# Autodesk Inventor assembly: for_bool
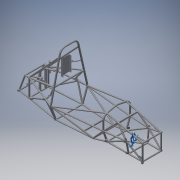
[picture p0: Inventor's stored thumbnail of the model, 180x180]
Saved by Autodesk Inventor 2018 (Build 220112000, 112)
## iProperties
Created: 2018-04-27
Part Number: for_bool
Material: 一般
Document SubType Name: Assembly
Designer: ku_sk
Author: ku_sk
## Documents named in this file (8)
- Z:\各班フォルダ\2018\ボディ\エアロ\Aero\KS-15\Fr.wing\parts\stay\parts\for_bool.iam
- Z:\各班フォルダ\2018\ボディ\エアロ\Aero\KS-15\Fr.wing\parts\stay\parts\frame.ipt
- Z:\各班フォルダ\2018\ボディ\エアロ\Aero\KS-15\Fr.wing\parts\stay\parts\bracket1(body).ipt
- Z:\各班フォルダ\2018\ボディ\エアロ\Aero\KS-15\Fr.wing\parts\stay\parts\bracket2(body).ipt
- Z:\各班フォルダ\2018\ボディ\エアロ\Aero\KS-15\Rr.wing\parts\stay\body-braket.ipt
- Z:\各班フォルダ\2018\ボディ\エアロ\Aero\KS-15\Fr.wing\parts\stay\parts\wire lead.ipt
- Z:\各班フォルダ\2018\ボディ\エアロ\Aero\KS-15\Fr.wing\parts\stay\parts\wire lead_MIR.ipt
- Z:\各班フォルダ\2018\ボディ\エアロ\Aero\KS-15\コスト用CAD\その他\3-Clamp.iam
## Components (7 placed, 7 different names)
1. frame:1 — メイト:1, メイト:2, メイト:3, メイト:6
2. bracket1(body):1 — 角度:2, 角度:3, フラッシュ:5, フラッシュ:6, フラッシュ:7
3. bracket2(body):1 — 角度:1, フラッシュ:9, フラッシュ:10, フラッシュ:11
4. body-braket:1 — フラッシュ:12, メイト:4, メイト:5
5. wire lead:1 — メイト:6
6. wire lead_MIR:1 — メイト:7, メイト:8
7. 3-Clamp:1 [sub-assembly] — メイト:7, メイト:8
## Relationships (18: Mate 8, Flush 7, Angle 3)
- メイト:1 [Mate]: frame:1
- メイト:2 [Mate]: frame:1
- メイト:3 [Mate]: frame:1
- 角度:1 [Angle] (0 deg): bracket2(body):1
- 角度:2 [Angle] (0 deg): bracket1(body):1
- 角度:3 [Angle] (0 deg): bracket1(body):1
- フラッシュ:5 [Flush] (1554.866 mm): bracket1(body):1
- フラッシュ:6 [Flush] (-179.5 mm): bracket1(body):1
- フラッシュ:7 [Flush] (-88.003 mm): bracket1(body):1
- フラッシュ:9 [Flush] (1526.124 mm): bracket2(body):1
- フラッシュ:10 [Flush] (-185.5 mm): bracket2(body):1
- フラッシュ:11 [Flush] (182.171 mm): bracket2(body):1
- フラッシュ:12 [Flush] (-182 mm): body-braket:1
- メイト:4 [Mate] (882.788 mm): body-braket:1
- メイト:5 [Mate] (-172.715 mm): body-braket:1
- メイト:6 [Mate]: frame:1 ↔ wire lead:1
- メイト:7 [Mate]: wire lead_MIR:1 ↔ 3-Clamp:1
- メイト:8 [Mate]: wire lead_MIR:1 ↔ 3-Clamp:1
